# Autodesk Inventor assembly: Assembly_Cube_Dichroic_Beamsplitter_multi_motorized_revolver_25x35_v3
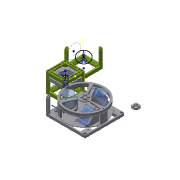
[picture p0: Inventor's stored thumbnail of the model, 180x180]
Saved by Autodesk Inventor 2019 (Build 230136000, 136)
## iProperties
Created: 2021-09-13
Part Number: Assembly_Cube_Dichroic_Beamsplitter_multi_motorized_revolver_25x35_v3
Document SubType Name: Assembly
Designer: diederichbenedict
Mass: 158.455 g
Surface Area: 1131.2 cm^2
Volume: 156.246 cm^3
Density: 1.01414 g/cm^3
Author: diederichbenedict
## Documents named in this file (12)
- C:\Users\Muriel\Downloads\UC2-MultiColour-master\UC2-MultiColour-master\INVENTOR\Workspace\Assembly_Cube_Dichroic_Beamsplitter_multi_motorized_revolver_25x35_v3.iam
- C:\Users\Muriel\Downloads\UC2-MultiColour-master\UC2-MultiColour-master\INVENTOR\Workspace\10_Cube_1x1_IM.ipt
- C:\Users\Muriel\Downloads\UC2-MultiColour-master\UC2-MultiColour-master\INVENTOR\Workspace\30_Cube_Insert_Filter_Revolver_Base_v3.ipt
- C:\Users\Muriel\Downloads\UC2-MultiColour-master\UC2-MultiColour-master\INVENTOR\Workspace\00_ballbearing_8mm.ipt
- C:\Users\Muriel\Downloads\UC2-MultiColour-master\UC2-MultiColour-master\INVENTOR\Workspace\30_Cube_Insert_Filter_Revolver_Wheel_v3.ipt
- C:\Users\Muriel\Downloads\UC2-MultiColour-master\UC2-MultiColour-master\INVENTOR\Workspace\30_Cube_Insert_Filter_Revolver_Filters_v3.iam
- C:\Users\Muriel\Downloads\UC2-MultiColour-master\UC2-MultiColour-master\INVENTOR\Workspace\30_Cube_Insert_Filter_Revolver_Wheel_Lid_v3.ipt
- C:\Users\Muriel\Downloads\UC2-MultiColour-master\UC2-MultiColour-master\INVENTOR\Workspace\30_Cube_Insert_Filter_Revolver_Lid.ipt
- C:\Users\Muriel\Downloads\UC2-MultiColour-master\UC2-MultiColour-master\INVENTOR\Workspace\Assembly_Cube_28byi_Motor_v3.iam
- C:\Users\Muriel\Downloads\UC2-MultiColour-master\UC2-MultiColour-master\INVENTOR\Workspace\10_Cube_Side_IM.ipt
- C:\Users\Muriel\Downloads\UC2-MultiColour-master\UC2-MultiColour-master\INVENTOR\Workspace\30_Cube_Insert_Filter_Revolver_Bearingmount_v3.ipt
- C:\Users\Muriel\Downloads\UC2-MultiColour-master\UC2-MultiColour-master\INVENTOR\Workspace\30_Cube_Insert_Filter_Revolver_Wheel_bearing_adapter_v3.ipt
## Components (18 placed, 11 different names)
1. 00_ballbearing_8mm:1 — Insert:1
2. 30_Cube_Insert_Filter_Revolver_Base_v3:1 — Insert:1
3. 30_Cube_Insert_Filter_Revolver_Wheel_v3:1 — Angle:3, Mate:30, Einfügen:2, Passend:33, Einfügen:5
4. 30_Cube_Insert_Filter_Revolver_Lid:1 — Passend:31, Fluchtend:14, Fluchtend:15, Fluchtend:16, Fluchtend:20, Passend:35, Einfügen:6
5. Assembly_Cube_28byi_Motor_v3:1 [sub-assembly] — Fluchtend:12, Fluchtend:13, Passend:32
6. 30_Cube_Insert_Filter_Revolver_Lid:2 — Fluchtend:12, Passend:31, Fluchtend:13, Passend:32, Fluchtend:14, Passend:34, Fluchtend:20, Passend:36
7. 30_Cube_Insert_Filter_Revolver_Wheel_Lid_v3:1 — Einfügen:2, Passend:33, Einfügen:4
8. 10_Cube_Side_IM:1 — Fluchtend:15, Fluchtend:16, Passend:34
9. 10_Cube_1x1_IM:1
10. 00_ballbearing_8mm:2 — Einfügen:3
11. 30_Cube_Insert_Filter_Revolver_Bearingmount_v3:1 — Passend:35, Passend:36, Einfügen:3
12. 30_Cube_Insert_Filter_Revolver_Bearingmount_v3:2
13. 00_ballbearing_8mm:3 — Einfügen:6
14. 30_Cube_Insert_Filter_Revolver_Wheel_bearing_adapter_v3:1 — Einfügen:4
15. 30_Cube_Insert_Filter_Revolver_Wheel_bearing_adapter_v3:2 — Einfügen:5
16. 30_Cube_Insert_Filter_Revolver_Filters_v3:1 [sub-assembly] — Mate:30
17. 30_Cube_Insert_Filter_Revolver_Filters_v3:2 [sub-assembly]
18. 30_Cube_Insert_Filter_Revolver_Filters_v3:3 [sub-assembly]
## Component patterns: (3 elements, first: 30_Cube_Insert_Filter_Revolver_Filters_v3:1)
## Relationships (20: Mate 7, Insert 6, Flush 6, Angle 1)
- Insert:1: 00_ballbearing_8mm:1 ↔ 30_Cube_Insert_Filter_Revolver_Base_v3:1
- Angle:3 (90 deg): 30_Cube_Insert_Filter_Revolver_Wheel_v3:1
- Mate:30: 30_Cube_Insert_Filter_Revolver_Wheel_v3:1 ↔ 30_Cube_Insert_Filter_Revolver_Filters_v3:1
- Fluchtend:12 [Flush]: Assembly_Cube_28byi_Motor_v3:1 ↔ 30_Cube_Insert_Filter_Revolver_Lid:2
- Passend:31 [Mate] (34 mm): 30_Cube_Insert_Filter_Revolver_Lid:1 ↔ 30_Cube_Insert_Filter_Revolver_Lid:2
- Fluchtend:13 [Flush]: Assembly_Cube_28byi_Motor_v3:1 ↔ 30_Cube_Insert_Filter_Revolver_Lid:2
- Passend:32 [Mate] (0.3 mm): Assembly_Cube_28byi_Motor_v3:1 ↔ 30_Cube_Insert_Filter_Revolver_Lid:2
- Fluchtend:14 [Flush]: 30_Cube_Insert_Filter_Revolver_Lid:1 ↔ 30_Cube_Insert_Filter_Revolver_Lid:2
- Einfügen:2 [Insert]: 30_Cube_Insert_Filter_Revolver_Wheel_v3:1 ↔ 30_Cube_Insert_Filter_Revolver_Wheel_Lid_v3:1
- Passend:33 [Mate]: 30_Cube_Insert_Filter_Revolver_Wheel_v3:1 ↔ 30_Cube_Insert_Filter_Revolver_Wheel_Lid_v3:1
- Fluchtend:15 [Flush]: 30_Cube_Insert_Filter_Revolver_Lid:1 ↔ 10_Cube_Side_IM:1
- Fluchtend:16 [Flush]: 30_Cube_Insert_Filter_Revolver_Lid:1 ↔ 10_Cube_Side_IM:1
- Passend:34 [Mate]: 30_Cube_Insert_Filter_Revolver_Lid:2 ↔ 10_Cube_Side_IM:1
- Fluchtend:20 [Flush]: 30_Cube_Insert_Filter_Revolver_Lid:1 ↔ 30_Cube_Insert_Filter_Revolver_Lid:2
- Passend:35 [Mate]: 30_Cube_Insert_Filter_Revolver_Lid:1 ↔ 30_Cube_Insert_Filter_Revolver_Bearingmount_v3:1
- Passend:36 [Mate]: 30_Cube_Insert_Filter_Revolver_Lid:2 ↔ 30_Cube_Insert_Filter_Revolver_Bearingmount_v3:1
- Einfügen:3 [Insert]: 00_ballbearing_8mm:2 ↔ 30_Cube_Insert_Filter_Revolver_Bearingmount_v3:1
- Einfügen:4 [Insert]: 30_Cube_Insert_Filter_Revolver_Wheel_Lid_v3:1 ↔ 30_Cube_Insert_Filter_Revolver_Wheel_bearing_adapter_v3:1
- Einfügen:5 [Insert]: 30_Cube_Insert_Filter_Revolver_Wheel_v3:1 ↔ 30_Cube_Insert_Filter_Revolver_Wheel_bearing_adapter_v3:2
- Einfügen:6 [Insert]: 30_Cube_Insert_Filter_Revolver_Lid:1 ↔ 00_ballbearing_8mm:3
